# Autodesk Inventor assembly: vexprowheel
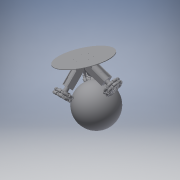
[picture p0: Inventor's stored thumbnail of the model, 180x180]
Saved by Autodesk Inventor 2016 (Build 200138000, 138)
## iProperties
Created: 2014-10-06
Part Number: vexprowheel
Description: STEP AP203
Document SubType Name: Assembly
Designer: Mack
Sending System: SolidWorks 2014
Preprocessor: SwSTEP 2.0
Title: 217-2584-STEP-20141006.STEP
Author: IFMI-VEX04
Revision Number: ANY
## Documents named in this file (5)
- C:\Users\Mack\Dropbox\2015-08 Fall\ECE459_Embedded-Systems\Project\models\vexprowheel.iam
- C:\Users\Mack\Dropbox\2015-08 Fall\ECE459_Embedded-Systems\Project\models\model.ipt
- C:\Users\Mack\Dropbox\2015-08 Fall\ECE459_Embedded-Systems\Project\models\WheelMotor.iam
- C:\Users\Mack\Dropbox\2015-08 Fall\ECE459_Embedded-Systems\Project\models\Basketball.ipt
- C:\Users\Mack\Dropbox\2015-08 Fall\ECE459_Embedded-Systems\Project\models\Base.ipt
## Components (6 placed, 4 different names)
1. model:1
2. WheelMotor:1 [sub-assembly] — Angle:1, Insert:5, Insert:6
3. WheelMotor:2 [sub-assembly] — Mate:2, Insert:2, Insert:3
4. WheelMotor:3 [sub-assembly] — Insert:4, Mate:3
5. Basketball:1 — Tangent:2
6. Base:1 — Mate:2, Insert:2, Insert:3, Insert:4, Mate:3, Insert:5, Insert:6, Tangent:2
## Relationships (11: Insert 6, Mate 3, Angle 1, Tangent 1)
- [Mate]: model:1 ↔ WheelMotor:1
- [Insert]: model:1 ↔ WheelMotor:1
- Angle:1 (225.1724 deg): WheelMotor:1
- Mate:2: WheelMotor:2 ↔ Base:1
- Insert:2: WheelMotor:2 ↔ Base:1
- Insert:3: WheelMotor:2 ↔ Base:1
- Insert:4: WheelMotor:3 ↔ Base:1
- Mate:3: WheelMotor:3 ↔ Base:1
- Insert:5: WheelMotor:1 ↔ Base:1
- Insert:6: WheelMotor:1 ↔ Base:1
- Tangent:2 (114.3 mm): Basketball:1 ↔ Base:1
